# Autodesk Inventor assembly: robot
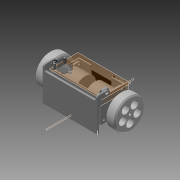
[picture p0: Inventor's stored thumbnail of the model, 180x180]
Saved by Autodesk Inventor 2015 (Build 190159000, 159)
## iProperties
Created: 2015-02-18
Part Number: robot
Document SubType Name: Assembly
Designer: jorge
Author: jorge
## Documents named in this file (14)
- \\psf\Home\Documents\proyectos\cybertech\sumo2015\sumo-2015\diseño3D\robot.iam
- \\psf\Home\Documents\proyectos\cybertech\sumo2015\sumo-2015\diseño3D\motor.ipt
- \\psf\Home\Documents\proyectos\cybertech\sumo2015\sumo-2015\diseño3D\base.ipt
- \\psf\Home\Documents\proyectos\cybertech\sumo2015\sumo-2015\diseño3D\king-max-1000-mah-lipo-battery-pack\Imported Components\bateria KingMax1000\bateria KingMax1000.ipt
- \\psf\Home\Documents\proyectos\cybertech\sumo2015\sumo-2015\diseño3D\arduino-nano-microcontroller-1\Imported Components\Arduino Mini ASSY\Arduino Mini ASSY.iam
- \\psf\Home\Documents\proyectos\cybertech\sumo2015\sumo-2015\diseño3D\mg90s-servo-1\Imported Components\MG90s_servo\MG90s_servo.ipt
- \\psf\Home\Documents\proyectos\cybertech\sumo2015\sumo-2015\diseño3D\tapa.ipt
- \\psf\Home\Documents\proyectos\cybertech\sumo2015\diseno\servo-horn-for-1-7-grams-ultra-micro-servo-1\Imported Components\servo_horn_1-7g\servo_horn_1-7g.ipt
- \\psf\Home\Documents\proyectos\cybertech\sumo2015\sumo-2015\diseño3D\llantasumo.ipt
- \\psf\Home\Documents\proyectos\cybertech\sumo2015\sumo-2015\diseño3D\pala.ipt
- \\psf\Home\Documents\proyectos\cybertech\sumo2015\sumo-2015\diseño3D\soporteDerecho.ipt
- \\psf\Home\Documents\proyectos\cybertech\sumo2015\sumo-2015\diseño3D\3mm-bearing-skf-623-rs-285-0790\Imported Components\3mm Bearing SKF 623 (RS 285-0790)\3mm Bearing SKF 623 (RS 285-0790).ipt
- \\psf\Home\Documents\proyectos\cybertech\sumo2015\sumo-2015\diseño3D\soporteIzq.ipt
- \\psf\Home\Documents\proyectos\cybertech\sumo2015\sumo-2015\diseño3D\castor.ipt
## Components (16 placed, 13 different names)
1. motor:1 — Cilíndrica:1
2. motor:2 — De rotación:1
3. base:1 — Rígido:3
4. bateria KingMax1000:1
5. Arduino Mini ASSY:1 [sub-assembly]
6. MG90s_servo:1
7. tapa:1 — Nivelación:1
8. servo_horn_1-7g:1
9. llantasumo:1 — De rotación:1
10. llantasumo:2 — Cilíndrica:1
11. pala:1
12. soporteDerecho:1 — Rígido:2, Cilíndrica:2
13. 3mm Bearing SKF 623 (RS 285-0790):1 — Rígido:2, Cilíndrica:2
14. 3mm Bearing SKF 623 (RS 285-0790):2
15. soporteIzq:1 — Nivelación:1
16. castor:1 — Rígido:3
## Relationships (6: CylindricalJoint 2, WeldJoint 2, RevoluteJoint 1, Flush 1)
- De rotación:1 [RevoluteJoint]: motor:2 ↔ llantasumo:1
- Cilíndrica:1 [CylindricalJoint]: motor:1 ↔ llantasumo:2
- Rígido:2 [WeldJoint]: soporteDerecho:1 ↔ 3mm Bearing SKF 623 (RS 285-0790):1
- Cilíndrica:2 [CylindricalJoint]: soporteDerecho:1 ↔ 3mm Bearing SKF 623 (RS 285-0790):1
- Nivelación:1 [Flush]: tapa:1 ↔ soporteIzq:1
- Rígido:3 [WeldJoint]: base:1 ↔ castor:1
